# Autodesk Inventor assembly: CHASSIS
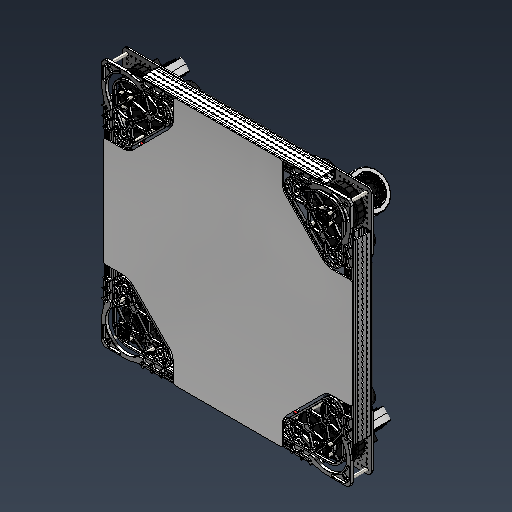
[picture p0: Inventor's stored thumbnail of the model, 512x512]
Saved by Autodesk Inventor 2026 (Build 300175050, 175E)
## iProperties
Created: 2026-01-19
Part Number: CHASSIS
Document SubType Name: Assembly
Designer: Jthib
Mass: 17091.3 g
Surface Area: 39405.1 cm^2
Volume: 6321.79 cm^3
Density: 2.70355 g/cm^3
Author: Jthib
## Documents named in this file (7)
- C:\Users\Jthib\Documents\GitHub\2026-Robot-Mechanical\Chassis\CHASSIS.iam
- C:\Users\Jthib\Documents\GitHub\2026-Robot-Mechanical\#1_CAD Library\SDS MK4i Swerve\ASSY,MK4i,HIGH,Swerve_Module.iam
- C:\Users\Jthib\Documents\GitHub\2026-Robot-Mechanical\Chassis\FRAME,MAXTUBE.ipt
- C:\Users\Jthib\Documents\GitHub\2026-Robot-Mechanical\#1_CAD Library\SDS MK4i Swerve\SDS Colson Wheel Kit.ipt
- C:\Users\Jthib\Documents\GitHub\2026-Robot-Mechanical\Chassis\PLATE,BELLYPAN.ipt
- C:\Users\Jthib\Documents\GitHub\2026-Robot-Mechanical\Chassis\PLATE,MOUNT,ELECTRONICS.ipt
- C:\Users\Jthib\Documents\GitHub\2026-Robot-Mechanical\#1_CAD Library\Motors\MOTOR,REV,NEO,V1-1.ipt
## Components (22 placed, 6 different names)
1. ASSY,MK4i,HIGH,Swerve_Module:1 [sub-assembly] — Mate:1, Mate:2, Mate:3, Mate:4, Mate:8, Mate:9, Insert:1, Insert:5, Insert:6, Insert:7, Insert:8
2. ASSY,MK4i,HIGH,Swerve_Module:2 [sub-assembly] — Mate:5, Mate:6, Mate:7, Mate:22, Mate:23, Mate:24, Insert:2, Insert:9, Insert:10, Insert:11, Insert:12
3. ASSY,MK4i,HIGH,Swerve_Module:3 [sub-assembly] — Mate:16, Mate:17, Mate:18, Mate:19, Mate:20, Mate:21, Insert:3, Flush:1, Flush:2, Insert:13, Insert:14, Insert:15, Insert:16
4. ASSY,MK4i,HIGH,Swerve_Module:4 [sub-assembly] — Mate:10, Mate:11, Mate:12, Mate:13, Mate:14, Mate:15, Insert:4, Insert:17, Insert:18, Insert:19, Insert:20
5. FRAME,MAXTUBE:1 — Mate:1, Mate:2, Mate:3, Mate:5, Mate:6, Mate:7, Symmetry:2
6. FRAME,MAXTUBE:2 — Mate:19, Mate:20, Mate:21, Mate:22, Mate:23, Symmetry:1
7. FRAME,MAXTUBE:3 — Mate:13, Mate:14, Mate:15, Mate:16, Mate:17, Mate:18, Mate:25, Flush:3, Symmetry:2
8. FRAME,MAXTUBE:4 — Mate:4, Mate:8, Mate:9, Mate:10, Mate:11, Mate:12, Flush:4, Symmetry:1
9. SDS Colson Wheel Kit:1 — Insert:2
10. SDS Colson Wheel Kit:2 — Insert:3
11. SDS Colson Wheel Kit:3 — Insert:4
12. SDS Colson Wheel Kit:4 — Insert:1
13. PLATE,BELLYPAN:1 — Flush:1, Flush:2
14. PLATE,MOUNT,ELECTRONICS:1 — Mate:25, Flush:3, Flush:4
15. MOTOR,REV,NEO,V1-1:1 — Insert:5, Insert:6
16. MOTOR,REV,NEO,V1-1:2 — Insert:7, Insert:8
17. MOTOR,REV,NEO,V1-1:3 — Insert:9, Insert:10
18. MOTOR,REV,NEO,V1-1:4 — Insert:11, Insert:12
19. MOTOR,REV,NEO,V1-1:5 — Insert:13, Insert:14
20. MOTOR,REV,NEO,V1-1:6 — Insert:15, Insert:16
21. MOTOR,REV,NEO,V1-1:7 — Insert:17, Insert:18
22. MOTOR,REV,NEO,V1-1:8 — Insert:19, Insert:20
## Relationships (51: Mate 25, Insert 20, Flush 4, Symmetry 2)
- Mate:1: ASSY,MK4i,HIGH,Swerve_Module:1 ↔ FRAME,MAXTUBE:1
- Mate:2: ASSY,MK4i,HIGH,Swerve_Module:1 ↔ FRAME,MAXTUBE:1
- Mate:3: ASSY,MK4i,HIGH,Swerve_Module:1 ↔ FRAME,MAXTUBE:1
- Mate:4: ASSY,MK4i,HIGH,Swerve_Module:1 ↔ FRAME,MAXTUBE:4
- Mate:5: ASSY,MK4i,HIGH,Swerve_Module:2 ↔ FRAME,MAXTUBE:1
- Mate:6: ASSY,MK4i,HIGH,Swerve_Module:2 ↔ FRAME,MAXTUBE:1
- Mate:7: ASSY,MK4i,HIGH,Swerve_Module:2 ↔ FRAME,MAXTUBE:1
- Mate:8: ASSY,MK4i,HIGH,Swerve_Module:1 ↔ FRAME,MAXTUBE:4
- Mate:9: ASSY,MK4i,HIGH,Swerve_Module:1 ↔ FRAME,MAXTUBE:4
- Mate:10: ASSY,MK4i,HIGH,Swerve_Module:4 ↔ FRAME,MAXTUBE:4
- Mate:11: ASSY,MK4i,HIGH,Swerve_Module:4 ↔ FRAME,MAXTUBE:4
- Mate:12: ASSY,MK4i,HIGH,Swerve_Module:4 ↔ FRAME,MAXTUBE:4
- Mate:13: ASSY,MK4i,HIGH,Swerve_Module:4 ↔ FRAME,MAXTUBE:3
- Mate:14: ASSY,MK4i,HIGH,Swerve_Module:4 ↔ FRAME,MAXTUBE:3
- Mate:15: ASSY,MK4i,HIGH,Swerve_Module:4 ↔ FRAME,MAXTUBE:3
- Mate:16: ASSY,MK4i,HIGH,Swerve_Module:3 ↔ FRAME,MAXTUBE:3
- Mate:17: ASSY,MK4i,HIGH,Swerve_Module:3 ↔ FRAME,MAXTUBE:3
- Mate:18: ASSY,MK4i,HIGH,Swerve_Module:3 ↔ FRAME,MAXTUBE:3
- Mate:19: ASSY,MK4i,HIGH,Swerve_Module:3 ↔ FRAME,MAXTUBE:2
- Mate:20: ASSY,MK4i,HIGH,Swerve_Module:3 ↔ FRAME,MAXTUBE:2
- Mate:21: ASSY,MK4i,HIGH,Swerve_Module:3 ↔ FRAME,MAXTUBE:2
- Mate:22: ASSY,MK4i,HIGH,Swerve_Module:2 ↔ FRAME,MAXTUBE:2
- Mate:23: ASSY,MK4i,HIGH,Swerve_Module:2 ↔ FRAME,MAXTUBE:2
- Mate:24 (95.25 mm): ASSY,MK4i,HIGH,Swerve_Module:2
- Insert:1: ASSY,MK4i,HIGH,Swerve_Module:1 ↔ SDS Colson Wheel Kit:4
- Insert:2: ASSY,MK4i,HIGH,Swerve_Module:2 ↔ SDS Colson Wheel Kit:1
- Insert:3: ASSY,MK4i,HIGH,Swerve_Module:3 ↔ SDS Colson Wheel Kit:2
- Insert:4: ASSY,MK4i,HIGH,Swerve_Module:4 ↔ SDS Colson Wheel Kit:3
- Flush:1: ASSY,MK4i,HIGH,Swerve_Module:3 ↔ PLATE,BELLYPAN:1
- Flush:2: ASSY,MK4i,HIGH,Swerve_Module:3 ↔ PLATE,BELLYPAN:1
- Mate:25: FRAME,MAXTUBE:3 ↔ PLATE,MOUNT,ELECTRONICS:1
- Flush:3: FRAME,MAXTUBE:3 ↔ PLATE,MOUNT,ELECTRONICS:1
- Flush:4: FRAME,MAXTUBE:4 ↔ PLATE,MOUNT,ELECTRONICS:1
- Symmetry:1: FRAME,MAXTUBE:2 ↔ FRAME,MAXTUBE:4
- Symmetry:2: FRAME,MAXTUBE:1 ↔ FRAME,MAXTUBE:3
- Insert:5: ASSY,MK4i,HIGH,Swerve_Module:1 ↔ MOTOR,REV,NEO,V1-1:1
- Insert:6: ASSY,MK4i,HIGH,Swerve_Module:1 ↔ MOTOR,REV,NEO,V1-1:1
- Insert:7: ASSY,MK4i,HIGH,Swerve_Module:1 ↔ MOTOR,REV,NEO,V1-1:2
- Insert:8: ASSY,MK4i,HIGH,Swerve_Module:1 ↔ MOTOR,REV,NEO,V1-1:2
- Insert:9: ASSY,MK4i,HIGH,Swerve_Module:2 ↔ MOTOR,REV,NEO,V1-1:3
- Insert:10: ASSY,MK4i,HIGH,Swerve_Module:2 ↔ MOTOR,REV,NEO,V1-1:3
- Insert:11: ASSY,MK4i,HIGH,Swerve_Module:2 ↔ MOTOR,REV,NEO,V1-1:4
- Insert:12: ASSY,MK4i,HIGH,Swerve_Module:2 ↔ MOTOR,REV,NEO,V1-1:4
- Insert:13: ASSY,MK4i,HIGH,Swerve_Module:3 ↔ MOTOR,REV,NEO,V1-1:5
- Insert:14: ASSY,MK4i,HIGH,Swerve_Module:3 ↔ MOTOR,REV,NEO,V1-1:5
- Insert:15: ASSY,MK4i,HIGH,Swerve_Module:3 ↔ MOTOR,REV,NEO,V1-1:6
- Insert:16: ASSY,MK4i,HIGH,Swerve_Module:3 ↔ MOTOR,REV,NEO,V1-1:6
- Insert:17: ASSY,MK4i,HIGH,Swerve_Module:4 ↔ MOTOR,REV,NEO,V1-1:7
- Insert:18: ASSY,MK4i,HIGH,Swerve_Module:4 ↔ MOTOR,REV,NEO,V1-1:7
- Insert:19: ASSY,MK4i,HIGH,Swerve_Module:4 ↔ MOTOR,REV,NEO,V1-1:8
- Insert:20: ASSY,MK4i,HIGH,Swerve_Module:4 ↔ MOTOR,REV,NEO,V1-1:8
